# Autodesk Inventor assembly: chwytak_core
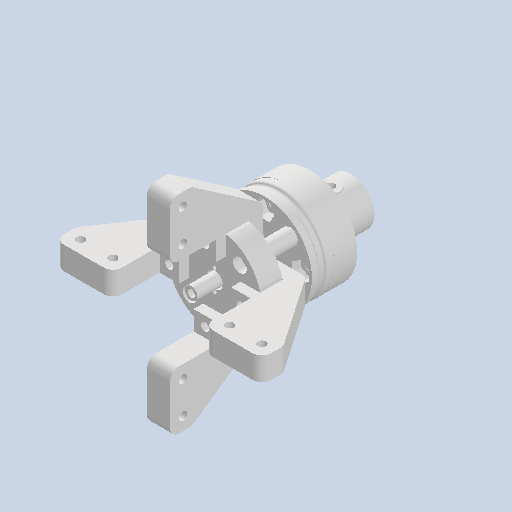
[picture p0: Inventor's stored thumbnail of the model, 512x512]
Saved by Autodesk Inventor 2023 (Build 270158000, 158)
## iProperties
Created: 2023-06-03
Part Number: chwytak_core
Document SubType Name: Assembly
Designer: Kamil
Author: Kamil
## Documents named in this file (7)
- C:\Users\Kamil\Desktop\KONARM_2\chwytak\chwytak_core.iam
- C:\Users\Kamil\Desktop\KONARM_2\chwytak\CircularStandOff.ipt
- C:\Users\Kamil\Desktop\KONARM_2\chwytak\ClawShoulder.ipt
- C:\Users\Kamil\Desktop\KONARM_2\chwytak\GripperBaseCircularLower.ipt
- C:\Users\Kamil\Desktop\KONARM_2\chwytak\GripperBaseCircularUpper.ipt
- C:\Users\Kamil\Desktop\KONARM_2\chwytak\ShaftToScrewCoupler.ipt
- C:\Users\Kamil\Desktop\KONARM_2\chwytak\uchwyt_na_oś.ipt
## Components (12 placed, 6 different names)
1. CircularStandOff:1 — Równoległe:5, Zestawiające:5, Zestawiające:7
2. ClawShoulder:1 — Zestawiające:9, Zestawiające:13, Równoległe:6
3. GripperBaseCircularLower:1 — Zestawiające:1, Zestawiające:2, Zestawiające:3, Zestawiające:4, Zestawiające:5, Zestawiające:18, Zestawiające:19
4. GripperBaseCircularUpper:1 — Zestawiające:6, Zestawiające:7, Zestawiające:8, Zestawiające:9, Zestawiające:10, Zestawiające:11, Zestawiające:12, Zestawiające:13, Zestawiające:14, Zestawiające:15, Zestawiające:16, Zestawiające:17, Równoległe:8
5. ClawShoulder:2 — Zestawiające:10, Równoległe:7, Zestawiające:16
6. ClawShoulder:3 — Zestawiające:11, Równoległe:7, Zestawiające:15
7. ClawShoulder:4 — Zestawiające:12, Zestawiające:14, Równoległe:6
8. CircularStandOff:2 — Równoległe:3, Równoległe:5, Zestawiające:4, Zestawiające:8
9. CircularStandOff:3 — Równoległe:4, Zestawiające:3, Zestawiające:6
10. CircularStandOff:4 — Równoległe:3, Równoległe:4, Zestawiające:1, Zestawiające:2
11. ShaftToScrewCoupler:1 — Zestawiające:17, Równoległe:8
12. uchwyt_na_oś:1 — Zestawiające:18, Zestawiające:19
## Relationships (25: Mate 19, Flush 6)
- Równoległe:3 [Flush]: CircularStandOff:2 ↔ CircularStandOff:4
- Równoległe:4 [Flush]: CircularStandOff:3 ↔ CircularStandOff:4
- Równoległe:5 [Flush]: CircularStandOff:1 ↔ CircularStandOff:2
- Zestawiające:1 [Mate]: GripperBaseCircularLower:1 ↔ CircularStandOff:4
- Zestawiające:2 [Mate]: GripperBaseCircularLower:1 ↔ CircularStandOff:4
- Zestawiające:3 [Mate]: GripperBaseCircularLower:1 ↔ CircularStandOff:3
- Zestawiające:4 [Mate]: GripperBaseCircularLower:1 ↔ CircularStandOff:2
- Zestawiające:5 [Mate]: CircularStandOff:1 ↔ GripperBaseCircularLower:1
- Zestawiające:6 [Mate]: GripperBaseCircularUpper:1 ↔ CircularStandOff:3
- Zestawiające:7 [Mate]: CircularStandOff:1 ↔ GripperBaseCircularUpper:1
- Zestawiające:8 [Mate]: GripperBaseCircularUpper:1 ↔ CircularStandOff:2
- Zestawiające:9 [Mate]: ClawShoulder:1 ↔ GripperBaseCircularUpper:1
- Zestawiające:10 [Mate]: GripperBaseCircularUpper:1 ↔ ClawShoulder:2
- Zestawiające:11 [Mate]: GripperBaseCircularUpper:1 ↔ ClawShoulder:3
- Zestawiające:12 [Mate]: GripperBaseCircularUpper:1 ↔ ClawShoulder:4
- Zestawiające:13 [Mate]: ClawShoulder:1 ↔ GripperBaseCircularUpper:1
- Zestawiające:14 [Mate]: GripperBaseCircularUpper:1 ↔ ClawShoulder:4
- Równoległe:6 [Flush]: ClawShoulder:1 ↔ ClawShoulder:4
- Równoległe:7 [Flush]: ClawShoulder:2 ↔ ClawShoulder:3
- Zestawiające:15 [Mate]: GripperBaseCircularUpper:1 ↔ ClawShoulder:3
- Zestawiające:16 [Mate]: GripperBaseCircularUpper:1 ↔ ClawShoulder:2
- Zestawiające:17 [Mate]: GripperBaseCircularUpper:1 ↔ ShaftToScrewCoupler:1
- Równoległe:8 [Flush] (0.5 mm): GripperBaseCircularUpper:1 ↔ ShaftToScrewCoupler:1
- Zestawiające:18 [Mate]: GripperBaseCircularLower:1 ↔ uchwyt_na_oś:1
- Zestawiające:19 [Mate]: GripperBaseCircularLower:1 ↔ uchwyt_na_oś:1
